# Autodesk Inventor assembly: CB185-120
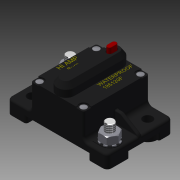
[picture p0: Inventor's stored thumbnail of the model, 180x180]
Saved by Autodesk Inventor 2016 (Build 200138000, 138)
## iProperties
Category: Electrical
Company: Autodesk Inc.
Shininess: 64.0
Length Units: 11272
Angle Units: 11279
Time Units: 11290
Mass Units: 11286
Length Display Precision: 3
Angle Display Precision: 2
Compacted: True
Part Number: CB185-120
Document SubType Name: Assembly
Created: 2015-12-10
Designer: Autodesk Inc.
Catalog Web Link: www.eaton.com/bussmanseries
Description: Circuit breaker
Vendor: Cooper Bussman
Density: 0.0
Volumn: 0.0
Area: 0.0
PropertySet Name: Model Information
Control State: 0
Master: False
Checked Out: False
Author: Autodesk Inc.
## Documents named in this file (8)
- E:\1073CAD\Robot2017\DriveTrain\Belly pan with electronics\FRC KOP 2016\Electrical\ELEC_CircuitBreaker_CB185-120.iam
- E:\1073CAD\Robot2017\DriveTrain\Belly pan with electronics\FRC KOP 2016\Electrical\Parts\BUSS-BASE.ipt
- E:\1073CAD\Robot2017\DriveTrain\Belly pan with electronics\FRC KOP 2016\Electrical\Parts\BUSS-COVER.ipt
- E:\1073CAD\Robot2017\DriveTrain\Belly pan with electronics\FRC KOP 2016\Electrical\Parts\BUSS-SAFTY-TRIP.ipt
- E:\1073CAD\Robot2017\DriveTrain\Belly pan with electronics\FRC KOP 2016\Electrical\Parts\BUSS-RIVET.ipt
- E:\1073CAD\Robot2017\DriveTrain\Belly pan with electronics\FRC KOP 2016\Electrical\Parts\BUSS-STUD-250X50.ipt
- E:\1073CAD\Robot2017\DriveTrain\Belly pan with electronics\FRC KOP 2016\Electrical\Parts\local.ANSI.1001.10.2.ipt
- E:\1073CAD\Robot2017\DriveTrain\Belly pan with electronics\FRC KOP 2016\Electrical\Parts\local.ANSI.1059.80.1.ipt
## Components (13 placed, 7 different names)
1. BUSS-BASE:1 — Mate:10, Flush:1, Mate:11, Flush:2, Insert:1, Insert:2
2. BUSS-COVER:1 — Mate:1, Mate:2, Mate:3, Mate:4, Mate:5, Mate:6, Mate:7, Mate:8, Mate:9, Mate:10
3. BUSS-SAFTY-TRIP:1 — Mate:1
4. BUSS-RIVET:1 — Mate:2, Mate:3
5. BUSS-RIVET:2 — Mate:4, Mate:7
6. BUSS-RIVET:3 — Mate:5, Mate:8
7. BUSS-RIVET:4 — Mate:6, Mate:9
8. BUSS-STUD-250X50:1 — Flush:1
9. BUSS-STUD-250X50:2 — Mate:11, Flush:2
10. Hex Nut - UNC (Regular Thread - Inch) 1/4 - 20:1 — Insert:4
11. Hex Nut - UNC (Regular Thread - Inch) 1/4 - 20:2 — Insert:3
12. External Tooth Lock Washer - Type A (Inch) 1/4. Carbon Steel:1 — Insert:1, Insert:4
13. External Tooth Lock Washer - Type A (Inch) 1/4. Carbon Steel:2 — Insert:2, Insert:3
## Relationships (17: Mate 11, Insert 4, Flush 2)
- Mate:1: BUSS-COVER:1 ↔ BUSS-SAFTY-TRIP:1
- Mate:2: BUSS-COVER:1 ↔ BUSS-RIVET:1
- Mate:3: BUSS-COVER:1 ↔ BUSS-RIVET:1
- Mate:4: BUSS-COVER:1 ↔ BUSS-RIVET:2
- Mate:5: BUSS-COVER:1 ↔ BUSS-RIVET:3
- Mate:6: BUSS-COVER:1 ↔ BUSS-RIVET:4
- Mate:7: BUSS-COVER:1 ↔ BUSS-RIVET:2
- Mate:8: BUSS-COVER:1 ↔ BUSS-RIVET:3
- Mate:9: BUSS-COVER:1 ↔ BUSS-RIVET:4
- Mate:10: BUSS-BASE:1 ↔ BUSS-COVER:1
- Flush:1: BUSS-BASE:1 ↔ BUSS-STUD-250X50:1
- Mate:11: BUSS-BASE:1 ↔ BUSS-STUD-250X50:2
- Flush:2: BUSS-BASE:1 ↔ BUSS-STUD-250X50:2
- Insert:1: BUSS-BASE:1 ↔ External Tooth Lock Washer - Type A (Inch) 1/4. Carbon Steel:1
- Insert:2: BUSS-BASE:1 ↔ External Tooth Lock Washer - Type A (Inch) 1/4. Carbon Steel:2
- Insert:3: Hex Nut - UNC (Regular Thread - Inch) 1/4 - 20:2 ↔ External Tooth Lock Washer - Type A (Inch) 1/4. Carbon Steel:2
- Insert:4: Hex Nut - UNC (Regular Thread - Inch) 1/4 - 20:1 ↔ External Tooth Lock Washer - Type A (Inch) 1/4. Carbon Steel:1
